# Autodesk Inventor assembly: A105EnsembleBoitierLaserV2
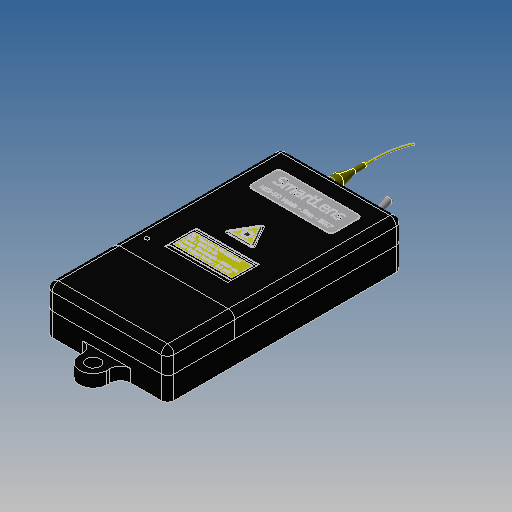
[picture p0: Inventor's stored thumbnail of the model, 512x512]
Saved by Autodesk Inventor 2019 (Build 230136000, 136)
## iProperties
Created: 2017-01-30
Part Number: A105EnsembleBoitierLaserV2
Document SubType Name: Assembly
Designer: serge.amoos
Author: serge.amoos
## Documents named in this file (13)
- I:\RaD\SI-ET\Projets\51346-SmartLens\inventor\FocalMeasure\A105EnsembleBoitierLaserV2.iam
- I:\RaD\SI-ET\Projets\51346-SmartLens\inventor\FocalMeasure\P301BoitierFond.ipt
- I:\RaD\SI-ET\Projets\51346-SmartLens\inventor\Imported Components\F111Batterie9V\F111Batterie9V.ipt
- I:\RaD\SI-ET\Projets\51346-SmartLens\inventor\FocalMeasure\F113PriseBatterie.ipt
- I:\RaD\SI-ET\Projets\51346-SmartLens\inventor\FocalMeasure\P121BoardLaser.ipt
- I:\RaD\SI-ET\Projets\51346-SmartLens\inventor\FocalMeasure\P302Radiateur.ipt
- I:\RaD\SI-ET\Projets\51346-SmartLens\inventor\Imported Components\F110LaserLP450\F110LaserLP450.iam
- I:\RaD\SI-ET\Projets\51346-SmartLens\inventor\FocalMeasure\F112Interrupteur.ipt
- I:\RaD\SI-ET\Projets\51346-SmartLens\inventor\FocalMeasure\P303CouvercleLaser.ipt
- I:\RaD\SI-ET\Projets\51346-SmartLens\inventor\FocalMeasure\P304CouvercleBatterie.ipt
- I:\RaD\SI-ET\Projets\51346-SmartLens\inventor\FocalMeasure\P305SigneLaser.ipt
- I:\RaD\SI-ET\Projets\51346-SmartLens\inventor\FocalMeasure\P306PlaqueLogo.ipt
- I:\RaD\SI-ET\Projets\51346-SmartLens\inventor\FocalMeasure\P308PlaqueThorlabs.ipt
## Components (12 placed, 12 different names)
1. P301BoitierFond:1 — Mate:3, Mate:6, Mate:7, Mate:9, Mate:10, Mate:11, Insert:2, Angle:3, Mate:12, Mate:13, Mate:14, Mate:15, Flush:1, Mate:16, Flush:2, Mate:18
2. F111Batterie9V:1 — Mate:1, Angle:1, Mate:2, Mate:3, Mate:12, Mate:13
3. F113PriseBatterie:1 — Mate:1, Angle:1, Mate:2
4. P121BoardLaser:1 — Mate:6, Mate:11, Mate:18
5. P302Radiateur:1 — Mate:7, Mate:9, Insert:1, Angle:2, Mate:10
6. F110LaserLP450:1 [sub-assembly] — Insert:1, Angle:2
7. F112Interrupteur:1 — Insert:2, Angle:3
8. P303CouvercleLaser:1 — Mate:14, Mate:15, Flush:1, Mate:17, Mate:19, Mate:20, Mate:21, Mate:22, Mate:23, Mate:24
9. P304CouvercleBatterie:1 — Mate:16, Flush:2, Mate:17
10. P305SigneLaser:1 — Mate:19
11. P306PlaqueLogo:1 — Mate:20, Mate:21, Mate:22
12. P308PlaqueThorlabs:1 — Mate:23, Mate:24
## Relationships (28: Mate 21, Angle 3, Insert 2, Flush 2)
- Mate:1: F111Batterie9V:1 ↔ F113PriseBatterie:1
- Angle:1 (0 deg): F111Batterie9V:1 ↔ F113PriseBatterie:1
- Mate:2 (2.5 mm): F111Batterie9V:1 ↔ F113PriseBatterie:1
- Mate:3: P301BoitierFond:1 ↔ F111Batterie9V:1
- Mate:6 (2 mm): P301BoitierFond:1 ↔ P121BoardLaser:1
- Mate:7: P301BoitierFond:1 ↔ P302Radiateur:1
- Mate:9: P301BoitierFond:1 ↔ P302Radiateur:1
- Insert:1: P302Radiateur:1 ↔ F110LaserLP450:1
- Angle:2 (90 deg): P302Radiateur:1 ↔ F110LaserLP450:1
- Mate:10 (0.1 mm): P301BoitierFond:1 ↔ P302Radiateur:1
- Mate:11 (2 mm): P301BoitierFond:1 ↔ P121BoardLaser:1
- Insert:2: P301BoitierFond:1 ↔ F112Interrupteur:1
- Angle:3 (0 deg): P301BoitierFond:1 ↔ F112Interrupteur:1
- Mate:12 (2 mm): P301BoitierFond:1 ↔ F111Batterie9V:1
- Mate:13 (1 mm): P301BoitierFond:1 ↔ F111Batterie9V:1
- Mate:14: P301BoitierFond:1 ↔ P303CouvercleLaser:1
- Mate:15: P301BoitierFond:1 ↔ P303CouvercleLaser:1
- Flush:1: P301BoitierFond:1 ↔ P303CouvercleLaser:1
- Mate:16: P301BoitierFond:1 ↔ P304CouvercleBatterie:1
- Flush:2: P301BoitierFond:1 ↔ P304CouvercleBatterie:1
- Mate:17: P303CouvercleLaser:1 ↔ P304CouvercleBatterie:1
- Mate:18 (2 mm): P301BoitierFond:1 ↔ P121BoardLaser:1
- Mate:19: P303CouvercleLaser:1 ↔ P305SigneLaser:1
- Mate:20: P303CouvercleLaser:1 ↔ P306PlaqueLogo:1
- Mate:21 (0.2 mm): P303CouvercleLaser:1 ↔ P306PlaqueLogo:1
- Mate:22 (0.2 mm): P303CouvercleLaser:1 ↔ P306PlaqueLogo:1
- Mate:23: P303CouvercleLaser:1 ↔ P308PlaqueThorlabs:1
- Mate:24: P303CouvercleLaser:1 ↔ P308PlaqueThorlabs:1
